# Autodesk Inventor assembly: Print
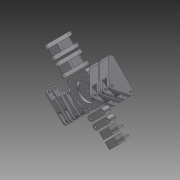
[picture p0: Inventor's stored thumbnail of the model, 180x180]
Saved by Autodesk Inventor 2011 SP2 (Build 150309200, 309)
## iProperties
Created: 2014-05-26
Part Number: Print
Document SubType Name: Assembly
Designer: Maurice Woods
Author: Maurice Woods
## Documents named in this file (8)
- C:\Users\Maurice\Documents\GitHub\strandbeest\Print.iam
- C:\Users\Maurice\Documents\GitHub\strandbeest\BDE.ipt
- C:\Users\Maurice\Documents\GitHub\strandbeest\F.ipt
- C:\Users\Maurice\Documents\GitHub\strandbeest\C.ipt
- C:\Users\Maurice\Documents\GitHub\strandbeest\GHI.ipt
- C:\Users\Maurice\Documents\GitHub\strandbeest\K.ipt
- C:\Users\Maurice\Documents\GitHub\strandbeest\MatingPlates.ipt
- C:\Users\Maurice\Documents\GitHub\strandbeest\J.ipt
## Components (13 placed, 7 different names)
1. BDE:1 — Mate:1, Mate:14, Mate:15, Mate:19, Tangent:1
2. F:1 — Mate:12, Mate:28, Mate:29, Tangent:4
3. C:1 — Mate:8, Mate:20, Mate:23, Mate:24
4. GHI:1 — Mate:4, Mate:17, Mate:18
5. K:1 — Mate:5, Mate:21, Mate:24, Mate:25
6. K:2 — Mate:6, Mate:22, Mate:25
7. MatingPlates:1 — Mate:13, Mate:14, Mate:16, Tangent:1, Tangent:2, Mate:26, Tangent:3, Mate:31, Mate:32, Tangent:6, Mate:33
8. C:2 — Mate:7, Mate:20, Mate:21, Mate:22, Mate:23, Mate:26, Tangent:3
9. F:2 — Mate:11, Mate:28, Tangent:5, Mate:31, Tangent:6
10. GHI:2 — Mate:3, Mate:16, Mate:17, Mate:18, Tangent:2
11. BDE:2 — Mate:2, Mate:15, Mate:19
12. J:1 — Mate:9, Mate:27, Mate:30
13. J:2 — Mate:10, Mate:27, Mate:29, Mate:30, Tangent:4, Tangent:5
## Relationships (39: Mate 33, Tangent 6)
- Mate:1: BDE:1
- Mate:2: BDE:2
- Mate:3: GHI:2
- Mate:4: GHI:1
- Mate:5: K:1
- Mate:6: K:2
- Mate:7: C:2
- Mate:8: C:1
- Mate:9: J:1
- Mate:10: J:2
- Mate:11: F:2
- Mate:12: F:1
- Mate:13: MatingPlates:1
- Mate:14 (3 mm): BDE:1 ↔ MatingPlates:1
- Mate:15 (3 mm): BDE:1 ↔ BDE:2
- Mate:16 (3 mm): MatingPlates:1 ↔ GHI:2
- Mate:17 (3 mm): GHI:1 ↔ GHI:2
- Mate:18: GHI:1 ↔ GHI:2
- Mate:19: BDE:1 ↔ BDE:2
- Tangent:1: BDE:1 ↔ MatingPlates:1
- Tangent:2: MatingPlates:1 ↔ GHI:2
- Mate:20: C:1 ↔ C:2
- Mate:21: K:1 ↔ C:2
- Mate:22: K:2 ↔ C:2
- Mate:23 (3 mm): C:1 ↔ C:2
- Mate:24 (3 mm): C:1 ↔ K:1
- Mate:25 (3 mm): K:1 ↔ K:2
- Mate:26 (3 mm): MatingPlates:1 ↔ C:2
- Tangent:3: MatingPlates:1 ↔ C:2
- Mate:27: J:1 ↔ J:2
- Mate:28 (3 mm): F:1 ↔ F:2
- Mate:29 (3 mm): F:1 ↔ J:2
- Mate:30 (3 mm): J:1 ↔ J:2
- Tangent:4: F:1 ↔ J:2
- Tangent:5: F:2 ↔ J:2
- Mate:31 (3 mm): MatingPlates:1 ↔ F:2
- Mate:32: MatingPlates:1
- Tangent:6: MatingPlates:1 ↔ F:2
- Mate:33: MatingPlates:1
